# Autodesk Inventor assembly: dish
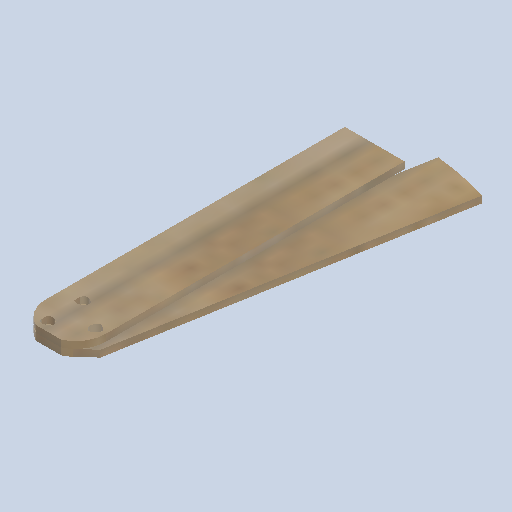
[picture p0: Inventor's stored thumbnail of the model, 512x512]
Saved by Autodesk Inventor 2024.1 (Build 281209000, 209)
## iProperties
Created: 2025-09-27
Part Number: dish
Document SubType Name: Assembly
Designer: hibik
Author: hibik
## Documents named in this file (3)
- C:\Users\hibik\Documents\Robomech\conveyer\belt\dish.iam
- C:\Users\hibik\Documents\Robomech\conveyer\belt\dish_upper.ipt
- C:\Users\hibik\Documents\Robomech\conveyer\belt\dish_under.ipt
## Components (2 placed, 2 different names)
1. dish_upper:1 — 挿入:1, 角度:1
2. dish_under:1 — 挿入:1, 角度:1
## Relationships (2: Insert 1, Angle 1)
- 挿入:1 [Insert]: dish_upper:1 ↔ dish_under:1
- 角度:1 [Angle] (0 deg): dish_upper:1 ↔ dish_under:1
